# Autodesk Inventor assembly: Frame 1780692296746
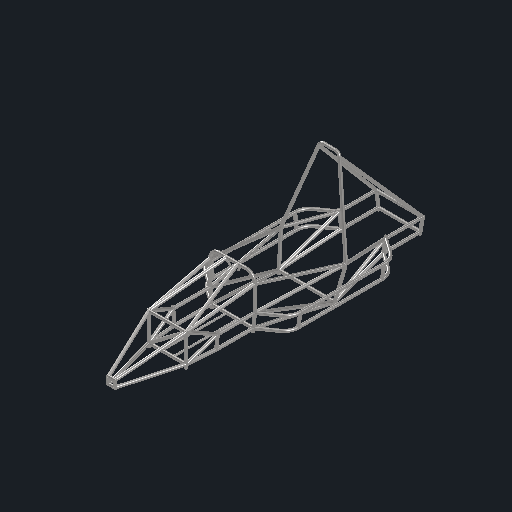
[picture p0: Inventor's stored thumbnail of the model, 512x512]
Saved by Autodesk Inventor 2026.1 (Build 301233000, 233)
## iProperties
_FrameDoc: Frame Assembly
_Version: 25.0.0
Created: 2026-06-05
Part Number: Frame 1780692296746
Document SubType Name: Assembly
Designer: tasle
Author: tasle
## Documents named in this file (71)
- C:\Users\share\OneDrive\Documents\Personal Projects\GOGO Kart\CAD\GOGO_KART_FSAE\FrameV2\Frame\Frame 1780692296746.iam
- C:\Users\share\OneDrive\Documents\Personal Projects\GOGO Kart\CAD\GOGO_KART_FSAE\FrameV2\Frame\Skeleton 1780692296747.ipt
- C:\Users\share\OneDrive\Documents\Personal Projects\GOGO Kart\CAD\GOGO_KART_FSAE\FrameV2\Frame\ANSI 1 x 0.179 1780692302546.ipt
- C:\Users\share\OneDrive\Documents\Personal Projects\GOGO Kart\CAD\GOGO_KART_FSAE\FrameV2\Frame\ANSI 1 x 0.179 1780692302574.ipt
- C:\Users\share\OneDrive\Documents\Personal Projects\GOGO Kart\CAD\GOGO_KART_FSAE\FrameV2\Frame\ANSI 1 x 0.179 1780692302595.ipt
- C:\Users\share\OneDrive\Documents\Personal Projects\GOGO Kart\CAD\GOGO_KART_FSAE\FrameV2\Frame\ANSI 1 x 0.179 1780692302622.ipt
- C:\Users\share\OneDrive\Documents\Personal Projects\GOGO Kart\CAD\GOGO_KART_FSAE\FrameV2\Frame\ANSI 1 x 0.179 1780692302650.ipt
- C:\Users\share\OneDrive\Documents\Personal Projects\GOGO Kart\CAD\GOGO_KART_FSAE\FrameV2\Frame\ANSI 1 x 0.179 1780692302672.ipt
- C:\Users\share\OneDrive\Documents\Personal Projects\GOGO Kart\CAD\GOGO_KART_FSAE\FrameV2\Frame\ANSI 1 x 0.179 1780692302694.ipt
- C:\Users\share\OneDrive\Documents\Personal Projects\GOGO Kart\CAD\GOGO_KART_FSAE\FrameV2\Frame\ANSI 1 x 0.179 1780692302716.ipt
- C:\Users\share\OneDrive\Documents\Personal Projects\GOGO Kart\CAD\GOGO_KART_FSAE\FrameV2\Frame\ANSI 1 x 0.179 1780692302739.ipt
- C:\Users\share\OneDrive\Documents\Personal Projects\GOGO Kart\CAD\GOGO_KART_FSAE\FrameV2\Frame\ANSI 1 x 0.179 1780692302759.ipt
- C:\Users\share\OneDrive\Documents\Personal Projects\GOGO Kart\CAD\GOGO_KART_FSAE\FrameV2\Frame\ANSI 1 x 0.179 1780692302779.ipt
- C:\Users\share\OneDrive\Documents\Personal Projects\GOGO Kart\CAD\GOGO_KART_FSAE\FrameV2\Frame\ANSI 1 x 0.179 1780692302799.ipt
- C:\Users\share\OneDrive\Documents\Personal Projects\GOGO Kart\CAD\GOGO_KART_FSAE\FrameV2\Frame\ANSI 1 x 0.179 1780692302820.ipt
- C:\Users\share\OneDrive\Documents\Personal Projects\GOGO Kart\CAD\GOGO_KART_FSAE\FrameV2\Frame\ANSI 1 x 0.179 1780692302840.ipt
- C:\Users\share\OneDrive\Documents\Personal Projects\GOGO Kart\CAD\GOGO_KART_FSAE\FrameV2\Frame\ANSI 1 x 0.179 1780692302880.ipt
- C:\Users\share\OneDrive\Documents\Personal Projects\GOGO Kart\CAD\GOGO_KART_FSAE\FrameV2\Frame\ANSI 1 x 0.179 1780692302901.ipt
- C:\Users\share\OneDrive\Documents\Personal Projects\GOGO Kart\CAD\GOGO_KART_FSAE\FrameV2\Frame\ANSI 1 x 0.179 1780692302942.ipt
- C:\Users\share\OneDrive\Documents\Personal Projects\GOGO Kart\CAD\GOGO_KART_FSAE\FrameV2\Frame\ANSI 1 x 0.179 1780692302962.ipt
- C:\Users\share\OneDrive\Documents\Personal Projects\GOGO Kart\CAD\GOGO_KART_FSAE\FrameV2\Frame\ANSI 1 x 0.179 1780692302983.ipt
- C:\Users\share\OneDrive\Documents\Personal Projects\GOGO Kart\CAD\GOGO_KART_FSAE\FrameV2\Frame\ANSI 1 x 0.179 1780692303004.ipt
- C:\Users\share\OneDrive\Documents\Personal Projects\GOGO Kart\CAD\GOGO_KART_FSAE\FrameV2\Frame\ANSI 1 x 0.179 1780692303025.ipt
- C:\Users\share\OneDrive\Documents\Personal Projects\GOGO Kart\CAD\GOGO_KART_FSAE\FrameV2\Frame\ANSI 1 x 0.179 1780692303065.ipt
- C:\Users\share\OneDrive\Documents\Personal Projects\GOGO Kart\CAD\GOGO_KART_FSAE\FrameV2\Frame\ANSI 1 x 0.179 1780692303109.ipt
- C:\Users\share\OneDrive\Documents\Personal Projects\GOGO Kart\CAD\GOGO_KART_FSAE\FrameV2\Frame\ANSI 1 x 0.179 1780692303131.ipt
- C:\Users\share\OneDrive\Documents\Personal Projects\GOGO Kart\CAD\GOGO_KART_FSAE\FrameV2\Frame\ANSI 1 x 0.179 1780692303282.ipt
- C:\Users\share\OneDrive\Documents\Personal Projects\GOGO Kart\CAD\GOGO_KART_FSAE\FrameV2\Frame\ANSI 1 x 0.179 1780692303302.ipt
- C:\Users\share\OneDrive\Documents\Personal Projects\GOGO Kart\CAD\GOGO_KART_FSAE\FrameV2\Frame\ANSI 1 x 0.179 1780692303344.ipt
- C:\Users\share\OneDrive\Documents\Personal Projects\GOGO Kart\CAD\GOGO_KART_FSAE\FrameV2\Frame\ANSI 1 x 0.179 1780692303426.ipt
- C:\Users\share\OneDrive\Documents\Personal Projects\GOGO Kart\CAD\GOGO_KART_FSAE\FrameV2\Frame\ANSI 1 x 0.179 1780692303471.ipt
- C:\Users\share\OneDrive\Documents\Personal Projects\GOGO Kart\CAD\GOGO_KART_FSAE\FrameV2\Frame\ANSI 1 x 0.179 1780692303492.ipt
- C:\Users\share\OneDrive\Documents\Personal Projects\GOGO Kart\CAD\GOGO_KART_FSAE\FrameV2\Frame\ANSI 1 x 0.179 1780692303687.ipt
- C:\Users\share\OneDrive\Documents\Personal Projects\GOGO Kart\CAD\GOGO_KART_FSAE\FrameV2\Frame\ANSI 1 x 0.179 1780692303707.ipt
- C:\Users\share\OneDrive\Documents\Personal Projects\GOGO Kart\CAD\GOGO_KART_FSAE\FrameV2\Frame\ANSI 1 x 0.179 1780692303816.ipt
- C:\Users\share\OneDrive\Documents\Personal Projects\GOGO Kart\CAD\GOGO_KART_FSAE\FrameV2\Frame\ANSI 1 x 0.179 1780692303838.ipt
- C:\Users\share\OneDrive\Documents\Personal Projects\GOGO Kart\CAD\GOGO_KART_FSAE\FrameV2\Frame\ANSI 1 x 0.179 1780692303858.ipt
- C:\Users\share\OneDrive\Documents\Personal Projects\GOGO Kart\CAD\GOGO_KART_FSAE\FrameV2\Frame\ANSI 1 x 0.179 1780692303879.ipt
- C:\Users\share\OneDrive\Documents\Personal Projects\GOGO Kart\CAD\GOGO_KART_FSAE\FrameV2\Frame\ANSI 1 x 0.179 1780692303920.ipt
- C:\Users\share\OneDrive\Documents\Personal Projects\GOGO Kart\CAD\GOGO_KART_FSAE\FrameV2\Frame\ANSI 1 x 0.179 1780692303940.ipt
- C:\Users\share\OneDrive\Documents\Personal Projects\GOGO Kart\CAD\GOGO_KART_FSAE\FrameV2\Frame\ANSI 1 x 0.179 1780692303966.ipt
- C:\Users\share\OneDrive\Documents\Personal Projects\GOGO Kart\CAD\GOGO_KART_FSAE\FrameV2\Frame\ANSI 1 x 0.179 1780692304008.ipt
- C:\Users\share\OneDrive\Documents\Personal Projects\GOGO Kart\CAD\GOGO_KART_FSAE\FrameV2\Frame\ANSI 1 x 0.179 1780692304091.ipt
- C:\Users\share\OneDrive\Documents\Personal Projects\GOGO Kart\CAD\GOGO_KART_FSAE\FrameV2\Frame\ANSI 1 x 0.179 1780692304111.ipt
- C:\Users\share\OneDrive\Documents\Personal Projects\GOGO Kart\CAD\GOGO_KART_FSAE\FrameV2\Frame\ANSI 1 x 0.179 1780692304131.ipt
- C:\Users\share\OneDrive\Documents\Personal Projects\GOGO Kart\CAD\GOGO_KART_FSAE\FrameV2\Frame\ANSI 1 x 0.179 1780692304151.ipt
- C:\Users\share\OneDrive\Documents\Personal Projects\GOGO Kart\CAD\GOGO_KART_FSAE\FrameV2\Frame\ANSI 1 x 0.179 1780692304297.ipt
- C:\Users\share\OneDrive\Documents\Personal Projects\GOGO Kart\CAD\GOGO_KART_FSAE\FrameV2\Frame\ANSI 1 x 0.179 1780692304340.ipt
- C:\Users\share\OneDrive\Documents\Personal Projects\GOGO Kart\CAD\GOGO_KART_FSAE\FrameV2\Frame\ANSI 1 x 0.179 1780692304362.ipt
- C:\Users\share\OneDrive\Documents\Personal Projects\GOGO Kart\CAD\GOGO_KART_FSAE\FrameV2\Frame\ANSI 1 x 0.179 1780692304384.ipt
- C:\Users\share\OneDrive\Documents\Personal Projects\GOGO Kart\CAD\GOGO_KART_FSAE\FrameV2\Frame\ANSI 1 x 0.179 1780692304405.ipt
- C:\Users\share\OneDrive\Documents\Personal Projects\GOGO Kart\CAD\GOGO_KART_FSAE\FrameV2\Frame\ANSI 1 x 0.179 1780692304425.ipt
- C:\Users\share\OneDrive\Documents\Personal Projects\GOGO Kart\CAD\GOGO_KART_FSAE\FrameV2\Frame\ANSI 1 x 0.179 1780692304445.ipt
- C:\Users\share\OneDrive\Documents\Personal Projects\GOGO Kart\CAD\GOGO_KART_FSAE\FrameV2\Frame\ANSI 1 x 0.179 1780692304465.ipt
- C:\Users\share\OneDrive\Documents\Personal Projects\GOGO Kart\CAD\GOGO_KART_FSAE\FrameV2\Frame\ANSI 1 x 0.179 1780692304485.ipt
- C:\Users\share\OneDrive\Documents\Personal Projects\GOGO Kart\CAD\GOGO_KART_FSAE\FrameV2\Frame\ANSI 1 x 0.179 1780692304506.ipt
- C:\Users\share\OneDrive\Documents\Personal Projects\GOGO Kart\CAD\GOGO_KART_FSAE\FrameV2\Frame\ANSI 1 x 0.179 1780692304526.ipt
- C:\Users\share\OneDrive\Documents\Personal Projects\GOGO Kart\CAD\GOGO_KART_FSAE\FrameV2\Frame\ANSI 1 x 0.179 1780692304546.ipt
- C:\Users\share\OneDrive\Documents\Personal Projects\GOGO Kart\CAD\GOGO_KART_FSAE\FrameV2\Frame\ANSI 1 x 0.179 1780692304587.ipt
- C:\Users\share\OneDrive\Documents\Personal Projects\GOGO Kart\CAD\GOGO_KART_FSAE\FrameV2\Frame\ANSI 1 x 0.179 1782332076807.ipt
- C:\Users\share\OneDrive\Documents\Personal Projects\GOGO Kart\CAD\GOGO_KART_FSAE\FrameV2\Frame\ANSI 1 x 0.179 1782332200115.ipt
- C:\Users\share\OneDrive\Documents\Personal Projects\GOGO Kart\CAD\GOGO_KART_FSAE\FrameV2\Frame\ANSI 1 x 0.179 1782332294883.ipt
- C:\Users\share\OneDrive\Documents\Personal Projects\GOGO Kart\CAD\GOGO_KART_FSAE\FrameV2\Frame\ANSI 1 x 0.179 1782332350122.ipt
- C:\Users\share\OneDrive\Documents\Personal Projects\GOGO Kart\CAD\GOGO_KART_FSAE\FrameV2\Frame\ANSI 1 x 0.179 1782332425793.ipt
- C:\Users\share\OneDrive\Documents\Personal Projects\GOGO Kart\CAD\GOGO_KART_FSAE\FrameV2\Frame\ANSI 1 x 0.179 1782332467531.ipt
- C:\Users\share\OneDrive\Documents\Personal Projects\GOGO Kart\CAD\GOGO_KART_FSAE\FrameV2\Frame\ANSI 1 x 0.179 1782334188549.ipt
- C:\Users\share\OneDrive\Documents\Personal Projects\GOGO Kart\CAD\GOGO_KART_FSAE\FrameV2\Frame\ANSI 1 x 0.179 1782334250193.ipt
- C:\Users\share\OneDrive\Documents\Personal Projects\GOGO Kart\CAD\GOGO_KART_FSAE\FrameV2\Frame\ANSI 1_2 x 0.109 1783344969371.ipt
- C:\Users\share\OneDrive\Documents\Personal Projects\GOGO Kart\CAD\GOGO_KART_FSAE\FrameV2\Frame\ANSI 1_2 x 0.109 1783344969395.ipt
- C:\Users\share\OneDrive\Documents\Personal Projects\GOGO Kart\CAD\GOGO_KART_FSAE\FrameV2\Frame\ANSI 1_2 x 0.109 1783352366176.ipt
- C:\Users\share\OneDrive\Documents\Personal Projects\GOGO Kart\CAD\GOGO_KART_FSAE\FrameV2\Frame\ANSI 1_2 x 0.109 1783352366199.ipt
## Components (70 placed, 32 different names)
1. Reference Skeleton
2. ANSI 1 x 0.179 - 26.119:1
3. ANSI 1 x 0.179 - 24.499:1
4. ANSI 1 x 0.179 - 26.119:2
5. ANSI 1 x 0.179 - 24.499:2
6. ANSI 1 x 0.179 - 4.076:1
7. ANSI 1 x 0.179 - 4.076:2
8. ANSI 1 x 0.179 - 4.076:3
9. ANSI 1 x 0.179 - 4.076:4
10. ANSI 1 x 0.179 - 15.748:1
11. ANSI 1 x 0.179 - 19.685:1
12. ANSI 1 x 0.179 - 13.971:1
13. ANSI 1 x 0.179 - 17.068:2
14. ANSI 1 x 0.179 - 13.971:2
15. ANSI 1 x 0.179 - 13.299:1
16. ANSI 1 x 0.179 - 13.299:2
17. ANSI 1 x 0.179 - 13.299:3
18. ANSI 1 x 0.179 - 6.935:1
19. ANSI 1 x 0.179 - 13.299:4
20. ANSI 1 x 0.179 - 29.409:1
21. ANSI 1 x 0.179 - 28.005:1
22. ANSI 1 x 0.179 - 28.005:2
23. ANSI 1 x 0.179 - 15.748:4
24. ANSI 1 x 0.179 - 6.935:3
25. ANSI 1 x 0.179 - 15.748:5
26. ANSI 1 x 0.179 - 17.717:1
27. ANSI 1 x 0.179 - 35.474:1
28. ANSI 1 x 0.179 - 34.727:1
29. ANSI 1 x 0.179 - 33.304:1
30. ANSI 1 x 0.179 - 31.985:1
31. ANSI 1 x 0.179 - 5.959:5
32. ANSI 1 x 0.179 - 5.959:6
33. ANSI 1 x 0.179 - 5.959:7
34. ANSI 1 x 0.179 - 35.474:2
35. ANSI 1 x 0.179 - 34.727:2
36. ANSI 1 x 0.179 - 33.304:2
37. ANSI 1 x 0.179 - 31.985:2
38. ANSI 1 x 0.179 - 25.963:1
39. ANSI 1 x 0.179 - 24.27:1
40. ANSI 1 x 0.179 - 21.285:1
41. ANSI 1 x 0.179 - 5.959:8
42. ANSI 1 x 0.179 - 7.987:9
43. ANSI 1 x 0.179 - 7.987:10
44. ANSI 1 x 0.179 - 25.963:2
45. ANSI 1 x 0.179 - 21.285:2
46. ANSI 1 x 0.179 - 45.719:1
47. ANSI 1 x 0.179 - 45.719:2
48. ANSI 1 x 0.179 - 15.748:8
49. ANSI 1 x 0.179 - 24.27:2
50. ANSI 1 x 0.179 - 23.622:1
51. ANSI 1 x 0.179 - 15.748:9
52. ANSI 1 x 0.179 - 7.766:11
53. ANSI 1 x 0.179 - 17.717:2
54. ANSI 1 x 0.179 - 21.243:2
55. ANSI 1 x 0.179 - 15.748:10
56. ANSI 1 x 0.179 - 15.748:11
57. ANSI 1 x 0.179 - 7.766:12
58. ANSI 1 x 0.179 - 29.409:1
59. ANSI 1 x 0.179 - 107.538:1
60. ANSI 1 x 0.179 - 59.522:1
61. ANSI 1 x 0.179 - 63.754:1
62. ANSI 1 x 0.179 - 63.754:2
63. ANSI 1 x 0.179 - 63.754:3
64. ANSI 1 x 0.179 - 63.754:4
65. ANSI 1 x 0.179 - 27.6:1
66. ANSI 1 x 0.179 - 27.6:2
67. ANSI 1/2 x 0.109 - 26.541:1
68. ANSI 1/2 x 0.109 - 26.541:2
69. ANSI 1/2 x 0.109 - 3.643:1
70. ANSI 1/2 x 0.109 - 3.643:2
## Relationships (1: Flush 1)
- Flush:1 (1450 mm)
